# Autodesk Inventor assembly: Neopixels
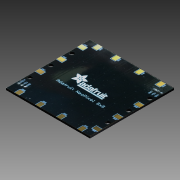
[picture p0: Inventor's stored thumbnail of the model, 180x180]
Saved by Autodesk Inventor 2014 (Build 180170000, 170)
## iProperties
Created: 2014-04-19
Part Number: Neopixels
Document SubType Name: Assembly
Designer: Ben
Author: Ben
## Documents named in this file (3)
- C:\Users\Ben Whiteside\SkyDrive\MNT\Micromoulding\Autocad Drawings\MakerStuff\Neopixels\Neopixels.iam
- C:\Users\Ben Whiteside\SkyDrive\MNT\Micromoulding\Autocad Drawings\MakerStuff\Neopixels\8x8 board.ipt
- C:\Users\Ben Whiteside\SkyDrive\MNT\Micromoulding\Autocad Drawings\MakerStuff\Neopixels\led.ipt
## Components (65 placed, 2 different names)
1. 8x8 board:1 — Flush:1, Flush:2, Mate:1
2. led:1 — Flush:1, Flush:2, Mate:1
3. led:2
4. led:3
5. led:4
6. led:5
7. led:6
8. led:7
9. led:8
10. led:9
11. led:10
12. led:11
13. led:12
14. led:13
15. led:14
16. led:15
17. led:16
18. led:17
19. led:18
20. led:19
21. led:20
22. led:21
23. led:22
24. led:23
25. led:24
26. led:25
27. led:26
28. led:27
29. led:28
30. led:29
31. led:30
32. led:31
33. led:32
34. led:33
35. led:34
36. led:35
37. led:36
38. led:37
39. led:38
40. led:39
41. led:40
42. led:41
43. led:42
44. led:43
45. led:44
46. led:45
47. led:46
48. led:47
49. led:48
50. led:49
51. led:50
52. led:51
53. led:52
54. led:53
55. led:54
56. led:55
57. led:56
58. led:57
59. led:58
60. led:59
61. led:60
62. led:61
63. led:62
64. led:63
65. led:64
## Component patterns: (64 elements, first: led:1)
## Relationships (3: Flush 2, Mate 1)
- Flush:1 (2 mm): 8x8 board:1 ↔ led:1
- Flush:2 (2 mm): 8x8 board:1 ↔ led:1
- Mate:1: 8x8 board:1 ↔ led:1
